# Autodesk Inventor assembly: Pauk
(part 2 of 2)
- Flush:21 (22.86 mm): Pertinaks:1 ↔ konektorservomotora:8
- Mate:143: Pertinaks:1 ↔ konektorservomotora:8
- Flush:22: konektorservomotora:8 ↔ konektorservomotora:9
- Flush:23 (25.4 mm): Pertinaks:1 ↔ konektorservomotora:9
- Mate:144: Pertinaks:1 ↔ konektorservomotora:9
- Flush:24: konektorservomotora:9 ↔ konektorservomotora:10
- Mate:145: Pertinaks:1 ↔ konektorservomotora:10
- Flush:25 (27.94 mm): Pertinaks:1 ↔ konektorservomotora:10
- Flush:26: konektorservomotora:10 ↔ konektorservomotora:11
- Flush:27 (2.54 mm): konektorservomotora:10 ↔ konektorservomotora:11
- Flush:28: konektorservomotora:10 ↔ konektorservomotora:11
- Flush:29: konektorservomotora:11 ↔ konektorservomotora:12
- Flush:30 (2.54 mm): konektorservomotora:11 ↔ konektorservomotora:12
- Flush:31: konektorservomotora:11 ↔ konektorservomotora:12
